# Autodesk Inventor assembly: HOT Assembly
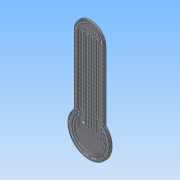
[picture p0: Inventor's stored thumbnail of the model, 180x180]
Saved by Autodesk Inventor 2013 (Build 170138000, 138)
## iProperties
Created: 2018-07-29
Part Number: HOT Assembly
Document SubType Name: Assembly
Designer: Jeff Vyduna
Author: Jeff Vyduna
## Documents named in this file (9)
- \\vmware-host\Shared Folders\Desktop\Bao sign 2018\CAD\1 HOT\HOT Assembly.iam
- \\vmware-host\Shared Folders\Desktop\Bao sign 2018\CAD\1 HOT\HOT Ply back.ipt
- \\vmware-host\Shared Folders\Desktop\Bao sign 2018\CAD\1 HOT\HOT SideBorder.ipt
- \\vmware-host\Shared Folders\Desktop\Bao sign 2018\CAD\1 HOT\HOT ThermoTop x2.ipt
- \\vmware-host\Shared Folders\Desktop\Bao sign 2018\CAD\1 HOT\Ply Leftover stock.ipt
- \\vmware-host\Shared Folders\Desktop\Bao sign 2018\CAD\1 HOT\Derived for CNC.ipt
- \\vmware-host\Shared Folders\Desktop\Bao sign 2018\CAD\1 HOT\HOT Thermo bulb outline L.ipt
- \\vmware-host\Shared Folders\Desktop\Bao sign 2018\CAD\1 HOT\HOT Thermo bulb outline B.ipt
- \\vmware-host\Shared Folders\Desktop\Bao sign 2018\CAD\1 HOT\HOT Thermo bulb outline R.ipt
## Components (9 placed, 8 different names)
1. HOT Ply back:1 — Flush:1, Flush:2, Flush:3, Flush:4, Insert:1, Mate:3, Insert:2, Flush:7, Flush:8, Mate:5, Mate:6, Insert:3, Insert:4, Mate:14
2. HOT SideBorder:1 — Flush:1, Flush:2, Mate:1, Mate:5, Mate:6, Mate:10, Mate:11, Mate:13
3. HOT ThermoTop x2:1 — Flush:3, Flush:4, Mate:2, Insert:1, Mate:3
4. HOT ThermoTop x2:2 — Mate:1, Mate:2, Insert:2
5. Ply Leftover stock:1 — Flush:7, Flush:8, Flush:9
6. Derived for CNC:1 — Flush:9
7. HOT Thermo bulb outline L:1 — Mate:12, Mate:13, Mate:14
8. HOT Thermo bulb outline B:1 — Insert:3, Mate:12
9. HOT Thermo bulb outline R:1 — Insert:4, Mate:10, Mate:11
## Relationships (21: Mate 10, Flush 7, Insert 4)
- Flush:1: HOT Ply back:1 ↔ HOT SideBorder:1
- Flush:2: HOT Ply back:1 ↔ HOT SideBorder:1
- Flush:3: HOT Ply back:1 ↔ HOT ThermoTop x2:1
- Flush:4: HOT Ply back:1 ↔ HOT ThermoTop x2:1
- Mate:1: HOT SideBorder:1 ↔ HOT ThermoTop x2:2
- Mate:2: HOT ThermoTop x2:1 ↔ HOT ThermoTop x2:2
- Insert:1: HOT Ply back:1 ↔ HOT ThermoTop x2:1
- Mate:3: HOT Ply back:1 ↔ HOT ThermoTop x2:1
- Insert:2: HOT Ply back:1 ↔ HOT ThermoTop x2:2
- Flush:7: HOT Ply back:1 ↔ Ply Leftover stock:1
- Flush:8: HOT Ply back:1 ↔ Ply Leftover stock:1
- Flush:9: Ply Leftover stock:1 ↔ Derived for CNC:1
- Mate:5: HOT Ply back:1 ↔ HOT SideBorder:1
- Mate:6: HOT Ply back:1 ↔ HOT SideBorder:1
- Insert:3: HOT Ply back:1 ↔ HOT Thermo bulb outline B:1
- Insert:4: HOT Ply back:1 ↔ HOT Thermo bulb outline R:1
- Mate:10: HOT SideBorder:1 ↔ HOT Thermo bulb outline R:1
- Mate:11: HOT SideBorder:1 ↔ HOT Thermo bulb outline R:1
- Mate:12: HOT Thermo bulb outline L:1 ↔ HOT Thermo bulb outline B:1
- Mate:13: HOT SideBorder:1 ↔ HOT Thermo bulb outline L:1
- Mate:14: HOT Ply back:1 ↔ HOT Thermo bulb outline L:1
